# Autodesk Inventor assembly: sPhenixTileTestStand
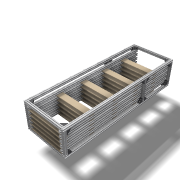
[picture p0: Inventor's stored thumbnail of the model, 180x180]
Saved by Autodesk Inventor 2017 (Build 210142000, 142)
## iProperties
Created: 2017-03-01
Part Number: sPhenixTileTestStand
Document SubType Name: Assembly
Designer: sawaiz
Author: sawaiz
## Documents named in this file (5)
- C:\Users\sawaiz\oneDrive\projects\sPhenixTileTestStand\sPhenixTileTestStand.iam
- C:\Users\sawaiz\oneDrive\projects\sPhenixTileTestStand\frame\frame.iam
- C:\Users\sawaiz\oneDrive\projects\sPhenixTileTestStand\plate\plate.iam
- C:\Users\sawaiz\Desktop\92605A229_NONMARRING FLAT POINT SET SCREW.ipt
- C:\Users\sawaiz\oneDrive\projects\sPhenixTileTestStand\sPhenixTileTestStand.xlsx
## Components (7 placed, 3 different names)
1. frame:1 [sub-assembly] — Mate:1, Mate:2, Angle:1
2. 92605A229_NONMARRING FLAT POINT SET SCREW:1
3. plate:1 [sub-assembly] — Mate:1, Mate:2, Angle:1
4. plate:2 [sub-assembly]
5. plate:3 [sub-assembly]
6. plate:4 [sub-assembly]
7. plate:5 [sub-assembly]
## Component patterns: (5 elements, first: plate:1)
## Relationships (3: Mate 2, Angle 1)
- Mate:1: frame:1 ↔ plate:1
- Mate:2 (3 mm): frame:1 ↔ plate:1
- Angle:1 (0 deg): frame:1 ↔ plate:1
## Named parameters: separation = 35 mm, numPanels = 5, plateWidth = 300 mm, plateDepth = 1000 mm, supportPlateThickness = 6.35 mm, supportPlateWidth = 50 mm, supportPlateFillet = 10 mm, centerVerticalRatio = 0.3
